# Autodesk Inventor assembly: TheLightWithinYou-Assembly-Threaded
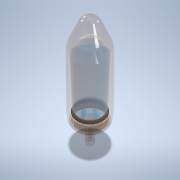
[picture p0: Inventor's stored thumbnail of the model, 180x180]
Saved by Autodesk Inventor 2021 (Build 250183000, 183)
## iProperties
Created: 2021-08-11
Part Number: TheLightWithinYou-Assembly-Threaded
Document SubType Name: Assembly
Designer: incep
Author: incep
## Documents named in this file (5)
- C:\Users\incep\Desktop\3D Printer Stuff\TheLightWithinYou\TheLightWithinYou-Assembly-Threaded.iam
- C:\Users\incep\Desktop\3D Printer Stuff\TheLightWithinYou\Bottom-Threaded.ipt
- C:\Users\incep\Desktop\3D Printer Stuff\TheLightWithinYou\Flashbulb.ipt
- C:\Users\incep\Desktop\3D Printer Stuff\TheLightWithinYou\Upper-Threaded.ipt
- C:\Users\incep\Desktop\3D Printer Stuff\TheLightWithinYou\R-22-O-ring.ipt
## Components (4 placed, 4 different names)
1. Bottom-Threaded:1 — Mate:1, Mate:2, Mate:3, Mate:4, Mate:5, Mate:6
2. Flashbulb:1 — Mate:1, Mate:2, Mate:3
3. Upper-Threaded:1 — Mate:5, Mate:6
4. R-22-O-ring:1 — Mate:4
## Relationships (6: Mate 6)
- Mate:1: Bottom-Threaded:1 ↔ Flashbulb:1
- Mate:2: Bottom-Threaded:1 ↔ Flashbulb:1
- Mate:3: Bottom-Threaded:1 ↔ Flashbulb:1
- Mate:4: Bottom-Threaded:1 ↔ R-22-O-ring:1
- Mate:5: Bottom-Threaded:1 ↔ Upper-Threaded:1
- Mate:6: Bottom-Threaded:1 ↔ Upper-Threaded:1
